# Autodesk Inventor assembly: 48-0003
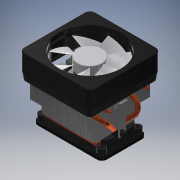
[picture p0: Inventor's stored thumbnail of the model, 180x180]
Saved by Autodesk Inventor 2018 (Build 220112000, 112)
## iProperties
Created: 2020-01-28
Part Number: 48-0003
Document SubType Name: Assembly
Designer: Bradley
Author: Bradley
## Documents named in this file (4)
- C:\Users\Bradley\Documents\GitHub\Resources\SupplierDocuments\48 - Hardware\48-0003\48-0003.iam
- C:\Users\Bradley\Documents\GitHub\Resources\SupplierDocuments\48 - Hardware\48-0003\BackBracket.ipt
- C:\Users\Bradley\Documents\GitHub\Resources\SupplierDocuments\48 - Hardware\48-0003\ClampHook.ipt
- C:\Users\Bradley\Documents\GitHub\Resources\SupplierDocuments\48 - Hardware\48-0003\Heatsink.ipt
## Components (4 placed, 3 different names)
1. BackBracket:1 — Insert:1, Insert:2, Insert:3, Insert:4
2. ClampHook:1 — Insert:1, Insert:2, Mate:1
3. ClampHook:2 — Insert:3, Insert:4
4. Heatsink:1 — Mate:1, Flush:1, Flush:2
## Relationships (7: Insert 4, Flush 2, Mate 1)
- Insert:1 (1.6 mm): BackBracket:1 ↔ ClampHook:1
- Insert:2 (1.6 mm): BackBracket:1 ↔ ClampHook:1
- Insert:3 (1.6 mm): BackBracket:1 ↔ ClampHook:2
- Insert:4 (1.6 mm): BackBracket:1 ↔ ClampHook:2
- Mate:1: ClampHook:1 ↔ Heatsink:1
- Flush:1: Heatsink:1
- Flush:2: Heatsink:1
